# Autodesk Inventor assembly: DC FAN 80 X 80 X 25
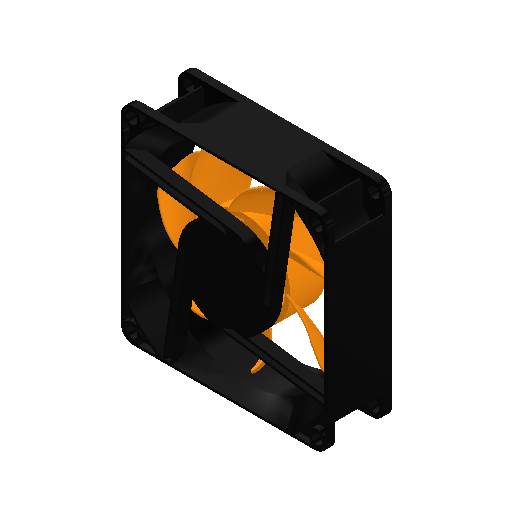
[picture p0: Inventor's stored thumbnail of the model, 512x512]
Saved by Autodesk Inventor 2026.2 (Build 302298010, 298A)
## iProperties
Created: 2017-06-06
Part Number: DC FAN 80 X 80 X 25
Description: STEP AP203
Document SubType Name: Assembly
Designer: danie
Sending System: SolidWorks 2016
Preprocessor: SwSTEP 2.0
Title: DC FAN 80 X 80 X 25.STEP
Revision Number: ANY
## Documents named in this file (3)
- C:\Users\danie\OneDrive\Documentos\Inventor\Arbol\V4\V4\dc-fan-80-x-80-x-25-mm-1.snapshot.1\DC FAN 80 X 80 X 25\DC FAN 80 X 80 X 25\DC FAN 80 X 80 X 25.iam
- C:\Users\danie\OneDrive\Documentos\Inventor\Arbol\V4\V4\dc-fan-80-x-80-x-25-mm-1.snapshot.1\DC FAN 80 X 80 X 25\DC FAN 80 X 80 X 25\FAN HOUSING 80 X 80 X 25.ipt
- C:\Users\danie\OneDrive\Documentos\Inventor\Arbol\V4\V4\dc-fan-80-x-80-x-25-mm-1.snapshot.1\DC FAN 80 X 80 X 25\DC FAN 80 X 80 X 25\FAN ROTOR 80 X 80 X 25.ipt
## Components (2 placed, 2 different names)
1. FAN HOUSING 80 X 80 X 25_1
2. FAN ROTOR 80 X 80 X 25_2 — Mate:1
## Relationships (1: Mate 1)
- Mate:1: FAN ROTOR 80 X 80 X 25_2
